# Autodesk Inventor assembly: Plato Carrete-doble B
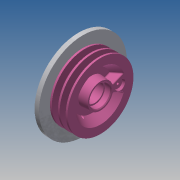
[picture p0: Inventor's stored thumbnail of the model, 180x180]
Saved by Autodesk Inventor 2017 (Build 210142000, 142)
## iProperties
Part Number: Plato Carrete-doble B
Material: Genérico
Document SubType Name: Assembly
Designer: FABLAB
Author: FABLAB
## Documents named in this file (3)
- C:\Users\FABLAB\Dropbox\E\Caja Motriz\transmision Engranajes\Plato Carrete-doble B.iam
- C:\Users\FABLAB\Dropbox\E\Caja Motriz\transmision Engranajes\Carrete Impreso.ipt
- C:\Users\FABLAB\Dropbox\E\Caja Motriz\transmision Engranajes\engrane acrílico C.ipt
## Components (2 placed, 2 different names)
1. Carrete Impreso:1 — Nivelación:1
2. engrane acrílico C:1 — Nivelación:1, Nivelación:2, Coincidencia:1
## Relationships (3: Flush 2, Mate 1)
- Nivelación:1 [Flush]: Carrete Impreso:1 ↔ engrane acrílico C:1
- Nivelación:2 [Flush]: engrane acrílico C:1
- Coincidencia:1 [Mate]: engrane acrílico C:1
